# Autodesk Inventor assembly: rectPaper
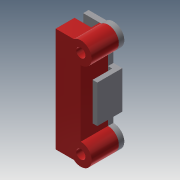
[picture p0: Inventor's stored thumbnail of the model, 180x180]
Saved by Autodesk Inventor 2019 (Build 230136000, 136)
## iProperties
Created: 2020-09-16
Part Number: rectPaper
Document SubType Name: Assembly
Designer: giacomo
Author: giacomo
## Documents named in this file (3)
- D:\Hobby\Inventor\Paper Clips\rectPaper.iam
- D:\Hobby\Inventor\Paper Clips\rectSopra.ipt
- D:\Hobby\Inventor\Paper Clips\rectSotto.ipt
## Components (2 placed, 2 different names)
1. rectSopra:1 — Mate:1, Mate:2, Mate:3
2. rectSotto:1 — Mate:1, Mate:2, Mate:3
## Relationships (3: Mate 3)
- Mate:1: rectSopra:1 ↔ rectSotto:1
- Mate:2: rectSopra:1 ↔ rectSotto:1
- Mate:3: rectSopra:1 ↔ rectSotto:1
